# Autodesk Inventor assembly: Manette_Chevaliers
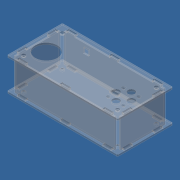
[picture p0: Inventor's stored thumbnail of the model, 180x180]
Saved by Autodesk Inventor 2015 SP2 (Build 190223200, 223)
## iProperties
Created: 2018-05-31
Part Number: Manette_Chevaliers
Project: Nom Projet
Description: Ens. Nom Ensemble
Document SubType Name: Assembly
Designer: Pierre-Olivier.SANDO
Author: Pierre-Olivier.SANDO
## Documents named in this file (6)
- Z:\COMMUN\4. Projets\1. Projets de semestre\P1704_Manette\2018\06_Dessins\Manette_Chevaliers\Manette_Chevaliers.iam
- Z:\COMMUN\4. Projets\1. Projets de semestre\P1704_Manette\2018\06_Dessins\Manette_Chevaliers\P1704_001_Toiture.ipt
- Z:\COMMUN\4. Projets\1. Projets de semestre\P1704_Manette\2018\06_Dessins\Manette_Chevaliers\P1704_002_Paroi_arrière.ipt
- Z:\COMMUN\4. Projets\1. Projets de semestre\P1704_Manette\2018\06_Dessins\Manette_Chevaliers\P1704_003_Paroi_avant.ipt
- Z:\COMMUN\4. Projets\1. Projets de semestre\P1704_Manette\2018\06_Dessins\Manette_Chevaliers\P1704_004_Paroi_latérale.ipt
- Z:\COMMUN\4. Projets\1. Projets de semestre\P1704_Manette\2018\06_Dessins\Manette_Chevaliers\P1704_005_Socle.ipt
## Components (6 placed, 5 different names)
1. P1704_004_Paroi_latérale:1 — Placage:4, Placage:5, Placage:6, Placage:13
2. P1704_001_Toiture:2 — Placage:13, Placage:14, Placage:15
3. P1704_002_Paroi_arrière:2 — Placage:7, Placage:8, Placage:9
4. P1704_003_Paroi_avant:2 — Placage:10, Placage:11, Placage:12, Placage:14, Placage:15
5. P1704_004_Paroi_latérale:2 — Placage:1, Placage:2, Placage:3
6. P1704_005_Socle:2 — Placage:1, Placage:2, Placage:3, Placage:4, Placage:5, Placage:6, Placage:7, Placage:8, Placage:9, Placage:10, Placage:11, Placage:12
## Relationships (15: Mate 15)
- Placage:1 [Mate]: P1704_004_Paroi_latérale:2 ↔ P1704_005_Socle:2
- Placage:2 [Mate]: P1704_004_Paroi_latérale:2 ↔ P1704_005_Socle:2
- Placage:3 [Mate]: P1704_004_Paroi_latérale:2 ↔ P1704_005_Socle:2
- Placage:4 [Mate]: P1704_004_Paroi_latérale:1 ↔ P1704_005_Socle:2
- Placage:5 [Mate]: P1704_004_Paroi_latérale:1 ↔ P1704_005_Socle:2
- Placage:6 [Mate]: P1704_004_Paroi_latérale:1 ↔ P1704_005_Socle:2
- Placage:7 [Mate]: P1704_002_Paroi_arrière:2 ↔ P1704_005_Socle:2
- Placage:8 [Mate]: P1704_002_Paroi_arrière:2 ↔ P1704_005_Socle:2
- Placage:9 [Mate]: P1704_002_Paroi_arrière:2 ↔ P1704_005_Socle:2
- Placage:10 [Mate]: P1704_003_Paroi_avant:2 ↔ P1704_005_Socle:2
- Placage:11 [Mate]: P1704_003_Paroi_avant:2 ↔ P1704_005_Socle:2
- Placage:12 [Mate]: P1704_003_Paroi_avant:2 ↔ P1704_005_Socle:2
- Placage:13 [Mate]: P1704_004_Paroi_latérale:1 ↔ P1704_001_Toiture:2
- Placage:14 [Mate]: P1704_001_Toiture:2 ↔ P1704_003_Paroi_avant:2
- Placage:15 [Mate]: P1704_001_Toiture:2 ↔ P1704_003_Paroi_avant:2
